# Autodesk Inventor assembly: Wheel_Assemblie
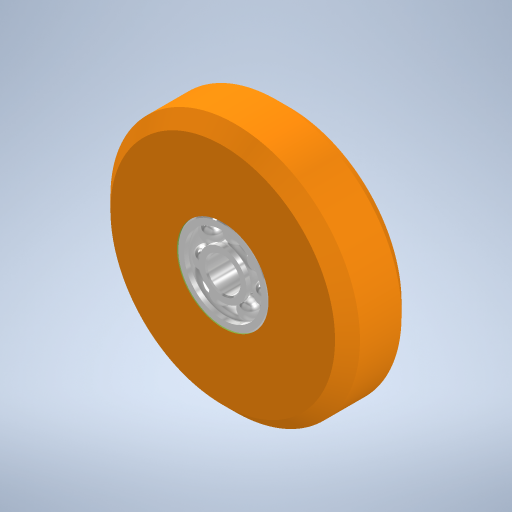
[picture p0: Inventor's stored thumbnail of the model, 512x512]
Saved by Autodesk Inventor 2023 (Build 270158000, 158)
## iProperties
Created: 2023-11-24
Part Number: Wheel_Assemblie
Document SubType Name: Assembly
Designer: danie
Author: danie
## Documents named in this file (3)
- D:\Diplomarbeit\3d-model\basis_roboter\low_rider_v2\custom_files\Wheel_Assemblie.iam
- D:\Diplomarbeit\3d-model\basis_roboter\low_rider_v2\custom_files\Wheel.ipt
- D:\Diplomarbeit\3d-model\basis_roboter\low_rider_v2\custom_files\Bearing.ipt
## Components (3 placed, 2 different names)
1. Wheel:1 — Rigid:1, Rigid:2
2. Bearing:1 — Rigid:1
3. Bearing:2 — Rigid:2
## Relationships (2: WeldJoint 2)
- Rigid:1 [WeldJoint]: Wheel:1 ↔ Bearing:1
- Rigid:2 [WeldJoint]: Wheel:1 ↔ Bearing:2
